# Autodesk Inventor assembly: ASY ANP 1490 FDS one way
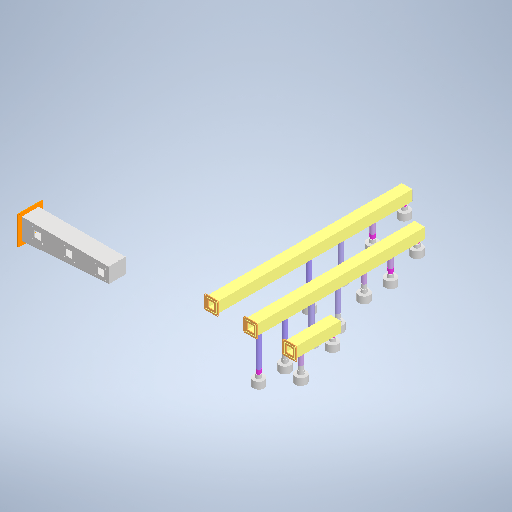
[picture p0: Inventor's stored thumbnail of the model, 512x512]
Saved by Autodesk Inventor 2025 (Build 290162010, 162A)
## iProperties
Created: 2025-07-22
Part Number: ASY ANP 1490 FDS one way
Document SubType Name: Assembly
Designer: admin
Stock Number: 20x40
Author: admin
## Documents named in this file (8)
- C:\Users\pokla\Documents\Inventor\ANP--Antipayuta\FDS 1400\ASY ANP 1490 FDS one way.iam
- C:\Users\pokla\Documents\Inventor\ANP--Antipayuta\FDS 1400\ANP 1422 BOTTOM FDS diameter way up.ipt
- C:\Users\pokla\Documents\Inventor\ANP--Antipayuta\FDS 1400\ANP 1421 FDS Diam way flange 1.ipt
- C:\Users\pokla\Documents\Inventor\ANP--Antipayuta\FDS 1400\ANP 1423 BOTTOM FDS diameter way down.ipt
- C:\Users\pokla\Documents\Inventor\ANP--Antipayuta\FDS 1400\ASY ANP 1425 FDS way 5.iam
- C:\Users\pokla\Documents\Inventor\ANP--Antipayuta\FDS 1400\ASY ANP 1426 FDS way 6.iam
- C:\Users\pokla\Documents\Inventor\ANP--Antipayuta\FDS 1400\ASY ANP 1427 FDS way 7.iam
- C:\Users\pokla\Documents\Inventor\ANP--Antipayuta\FDS 1400\ANP 1424 FDS diam way cup.ipt
## Components (7 placed, 7 different names)
1. ANP 1422 BOTTOM FDS diameter way up.ipt:1
2. ANP 1421 FDS Diam way flange 1.ipt:1
3. ANP 1423 BOTTOM FDS diameter way down.ipt:1 — Rigid:18
4. ASY ANP 1425 FDS way 5.iam:1 [sub-assembly]
5. ASY ANP 1426 FDS way 6.iam:1 [sub-assembly]
6. ASY ANP 1427 FDS way 7.iam:1 [sub-assembly]
7. ANP 1424 FDS diam way cup.ipt:1 — Rigid:18
## Relationships (7: Mate 3, Flush 3, WeldJoint 1)
- [Mate]: ANP 1422 BOTTOM FDS diameter way up.ipt:1 ↔ ANP 1421 FDS Diam way flange 1.ipt:1
- [Flush]: ANP 1422 BOTTOM FDS diameter way up.ipt:1 ↔ ANP 1421 FDS Diam way flange 1.ipt:1
- [Flush]: ANP 1422 BOTTOM FDS diameter way up.ipt:1 ↔ ANP 1421 FDS Diam way flange 1.ipt:1
- [Mate]: ANP 1421 FDS Diam way flange 1.ipt:1 ↔ ANP 1423 BOTTOM FDS diameter way down.ipt:1
- [Flush]: ANP 1421 FDS Diam way flange 1.ipt:1 ↔ ANP 1423 BOTTOM FDS diameter way down.ipt:1
- [Mate]: ANP 1422 BOTTOM FDS diameter way up.ipt:1 ↔ ANP 1423 BOTTOM FDS diameter way down.ipt:1
- Rigid:18 [WeldJoint]: ANP 1423 BOTTOM FDS diameter way down.ipt:1 ↔ ANP 1424 FDS diam way cup.ipt:1
